# Autodesk Inventor assembly: HbWrist
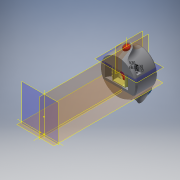
[picture p0: Inventor's stored thumbnail of the model, 180x180]
Saved by Autodesk Inventor 2017 (Build 210142000, 142)
## iProperties
Part Number: HbWrist
Material: 一般
Document SubType Name: Assembly
Designer: sktom
Author: sktom
## Documents named in this file (8)
- D:\OneDrive\ToDo_加工\@MAJ\STL69%inlength\wrist\HbWrist.iam
- D:\OneDrive\ToDo_加工\@MAJ\STL69%inlength\wrist\HBarmMountBase03ForChild.ipt
- D:\OneDrive\ToDo_加工\@MAJ\STL69%inlength\wrist\HBpronationLockPin02ForChild.ipt
- D:\OneDrive\ToDo_加工\@MAJ\STL69%inlength\wrist\HBlockPlateHolder02ForChild.ipt
- D:\OneDrive\ToDo_加工\@MAJ\STL69%inlength\wrist\HBejectorLever02ForChild.ipt
- D:\OneDrive\ToDo_加工\@MAJ\STL69%inlength\wrist\HBarmMount02ForChild.ipt
- D:\OneDrive\ToDo_加工\@MAJ\STL69%inlength\wrist\HBabductionLever02forChild.ipt
- D:\OneDrive\ToDo_加工\@MAJ\STL69%inlength\wrist\HBarmMountBaseCover03ForChild.ipt
## Components (7 placed, 7 different names)
1. HBarmMountBase03ForChild:1 — 挿入:1, 円柱状:1, フラッシュ:1, 円柱状:5, 挿入:2, 挿入:3
2. HBlockPlateHolder02ForChild:1 — 挿入:1
3. HBarmMount02ForChild:1 — 円柱状:2, 円柱状:7, メイト:1
4. HBpronationLockPin02ForChild:1 — 円柱状:5
5. HBejectorLever02ForChild:1 — 円柱状:2, 円柱状:6, 円柱状:7
6. HBabductionLever02forChild:1 — 円柱状:1, フラッシュ:1, 円柱状:6
7. HBarmMountBaseCover03ForChild:1 — 挿入:2, 挿入:3, メイト:1
## Relationships (10: CylindricalJoint 5, Insert 3, Flush 1, Mate 1)
- 挿入:1 [Insert]: HBarmMountBase03ForChild:1 ↔ HBlockPlateHolder02ForChild:1
- 円柱状:1 [CylindricalJoint]: HBarmMountBase03ForChild:1 ↔ HBabductionLever02forChild:1
- フラッシュ:1 [Flush]: HBarmMountBase03ForChild:1 ↔ HBabductionLever02forChild:1
- 円柱状:2 [CylindricalJoint]: HBarmMount02ForChild:1 ↔ HBejectorLever02ForChild:1
- 円柱状:5 [CylindricalJoint]: HBarmMountBase03ForChild:1 ↔ HBpronationLockPin02ForChild:1
- 円柱状:6 [CylindricalJoint]: HBejectorLever02ForChild:1 ↔ HBabductionLever02forChild:1
- 挿入:2 [Insert]: HBarmMountBase03ForChild:1 ↔ HBarmMountBaseCover03ForChild:1
- 挿入:3 [Insert]: HBarmMountBase03ForChild:1 ↔ HBarmMountBaseCover03ForChild:1
- 円柱状:7 [CylindricalJoint]: HBarmMount02ForChild:1 ↔ HBejectorLever02ForChild:1
- メイト:1 [Mate] (0.1 mm): HBarmMount02ForChild:1 ↔ HBarmMountBaseCover03ForChild:1
